# Autodesk Inventor assembly: 01 MAIN ASM Ender_3
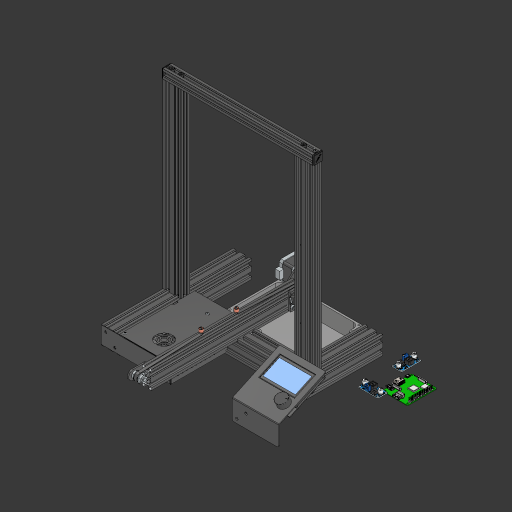
[picture p0: Inventor's stored thumbnail of the model, 512x512]
Saved by Autodesk Inventor 2023 (Build 270158000, 158)
## iProperties
Created: 2018-08-14
Part Number: 01 MAIN ASM Ender_3
Document SubType Name: Assembly
Designer: alber
Sending System: SolidWorks 2015
Last Author: Poseidon
Last Saved: 2018-08-17
Author: alber
## Documents named in this file (12)
- C:\Users\alber\Desktop\Files\Ender3-Upgrade\CAD\01 MAIN ASM Ender_3.iam
- C:\Users\alber\Desktop\Files\Ender3-Upgrade\CAD\ASM Frame.iam
- C:\Users\alber\Desktop\Files\Ender3-Upgrade\CAD\ASM X-Axis.iam
- C:\Users\alber\Desktop\Files\Ender3-Upgrade\CAD\ASM Y-Axis.iam
- C:\Users\alber\Desktop\Files\Ender3-Upgrade\CAD\ASM Z-Axis.iam
- C:\Users\alber\Desktop\Files\Ender3-Upgrade\CAD\ASM Display.iam
- C:\Users\alber\Desktop\Files\Ender3-Upgrade\CAD\ASM Electronic Enclosure.iam
- C:\Users\alber\Desktop\Files\Ender3-Upgrade\CAD\ASM Power Supply.iam
- C:\Users\alber\Desktop\Files\Ender3-Upgrade\CAD\RaspberryPi 3 A+.iam
- C:\Users\alber\Desktop\Files\Ender3-Upgrade\CAD\LM2596 DC to DC Buck Converter 3 A\converterLM2596.iam
- C:\Users\alber\Desktop\Files\Ender3-Upgrade\CAD\LED Bar.iam
- C:\Users\alber\Desktop\Files\Ender3-Upgrade\CAD\Back_Case.ipt
## Components (12 placed, 11 different names)
1. ASM Frame:1 [sub-assembly] — Mate:1, Mate:2, Mate:3, Mate:4, Mate:5, Mate:6, Mate:7, Flush:1
2. ASM X-Axis:1 [sub-assembly]
3. ASM Y-Axis:1 [sub-assembly]
4. ASM Z-Axis:1 [sub-assembly]
5. ASM Display:1 [sub-assembly]
6. ASM Electronic Enclosure:1 [sub-assembly]
7. ASM Power Supply:1 [sub-assembly]
8. RaspberryPi 3 A+:1 [sub-assembly]
9. converterLM2596:1 [sub-assembly]
10. converterLM2596:2 [sub-assembly]
11. LED Bar:1 [sub-assembly] — Mate:1, Mate:2, Mate:3, Mate:4, Mate:5, Mate:6, Mate:7
12. Back_Case:1 — Flush:1
## Relationships (8: Mate 7, Flush 1)
- Mate:1 (0.4 mm): ASM Frame:1 ↔ LED Bar:1
- Mate:2 (0.4 mm): ASM Frame:1 ↔ LED Bar:1
- Mate:3 (0.4 mm): ASM Frame:1 ↔ LED Bar:1
- Mate:4 (0.4 mm): ASM Frame:1 ↔ LED Bar:1
- Mate:5 (0.4 mm): ASM Frame:1 ↔ LED Bar:1
- Mate:6 (0.4 mm): ASM Frame:1 ↔ LED Bar:1
- Mate:7 (0.4 mm): ASM Frame:1 ↔ LED Bar:1
- Flush:1: ASM Frame:1 ↔ Back_Case:1
